# Autodesk Inventor assembly: Zusammenbau
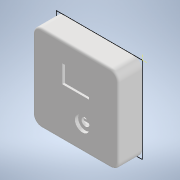
[picture p0: Inventor's stored thumbnail of the model, 180x180]
Saved by Autodesk Inventor 2022.2 (Build 262287000, 287)
## iProperties
Created: 2022-01-22
Part Number: Zusammenbau
Document SubType Name: Assembly
Designer: hpcwoess
Author: hpcwoess
## Documents named in this file (4)
- C:\QSync\3DPrints\Thermostat\Zusammenbau.iam
- C:\QSync\3DPrints\Thermostat\Clip.ipt
- C:\QSync\3DPrints\Thermostat\ClipUnten.ipt
- C:\QSync\3DPrints\Thermostat\Deckel.ipt
## Components (3 placed, 3 different names)
1. Clip:1 — Fluchtend:1, Passend:1, Fluchtend:2, Fluchtend:3, Fluchtend:4, Passend:2, Fluchtend:8
2. ClipUnten:1 — Fluchtend:1, Passend:1, Passend:2
3. Deckel:1 — Fluchtend:7, Fluchtend:8, Passend:3
## Relationships (9: Flush 6, Mate 3)
- Fluchtend:1 [Flush]: Clip:1 ↔ ClipUnten:1
- Passend:1 [Mate]: Clip:1 ↔ ClipUnten:1
- Fluchtend:2 [Flush]: Clip:1
- Fluchtend:3 [Flush]: Clip:1
- Fluchtend:4 [Flush]: Clip:1
- Passend:2 [Mate]: Clip:1 ↔ ClipUnten:1
- Fluchtend:7 [Flush]: Deckel:1
- Fluchtend:8 [Flush]: Clip:1 ↔ Deckel:1
- Passend:3 [Mate]: Deckel:1
